# Autodesk Inventor assembly: HighFlowCO2Laser
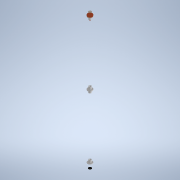
[picture p0: Inventor's stored thumbnail of the model, 180x180]
Saved by Autodesk Inventor 2020 (Build 240168000, 168)
## iProperties
Created: 2019-09-29
Part Number: HighFlowCO2Laser
Document SubType Name: Assembly
Designer: vmiguel
Author: vmiguel
## Documents named in this file (5)
- C:\Users\vmiguel\Documents\GitHub\HighFlowCO2Laser\HighFlowCO2Laser.iam
- C:\Users\vmiguel\Documents\GitHub\HighFlowCO2Laser\ZnSeWindow.ipt
- C:\Users\vmiguel\Documents\GitHub\HighFlowCO2Laser\GoldPlatedCopperMirror.ipt
- C:\Users\vmiguel\Documents\GitHub\HighFlowCO2Laser\TungstenFlange.ipt
- C:\Users\vmiguel\Documents\GitHub\HighFlowCO2Laser\CopperElectrode.ipt
## Components (7 placed, 4 different names)
1. ZnSeWindow:1 — Mate:1, Mate:8
2. GoldPlatedCopperMirror:1 — Mate:1
3. TungstenFlange:1 — Mate:5, Mate:6, Mate:8, Mate:9, Mate:13, Mate:14
4. TungstenFlange:2 — Mate:2, Mate:3, Mate:4, Mate:5, Mate:6, Mate:9, Mate:12
5. TungstenFlange:3 — Mate:2, Mate:3, Mate:4, Mate:10, Mate:11
6. TungstenFlange:4 — Mate:10, Mate:11, Mate:12
7. CopperElectrode:1 — Mate:13, Mate:14
## Relationships (13: Mate 13)
- Mate:1: ZnSeWindow:1 ↔ GoldPlatedCopperMirror:1
- Mate:2: TungstenFlange:2 ↔ TungstenFlange:3
- Mate:3: TungstenFlange:2 ↔ TungstenFlange:3
- Mate:4: TungstenFlange:2 ↔ TungstenFlange:3
- Mate:5: TungstenFlange:1 ↔ TungstenFlange:2
- Mate:6: TungstenFlange:1 ↔ TungstenFlange:2
- Mate:8: ZnSeWindow:1 ↔ TungstenFlange:1
- Mate:9 (500 mm): TungstenFlange:1 ↔ TungstenFlange:2
- Mate:10 (500 mm): TungstenFlange:3 ↔ TungstenFlange:4
- Mate:11: TungstenFlange:3 ↔ TungstenFlange:4
- Mate:12: TungstenFlange:2 ↔ TungstenFlange:4
- Mate:13: TungstenFlange:1 ↔ CopperElectrode:1
- Mate:14 (2 mm): TungstenFlange:1 ↔ CopperElectrode:1
